# Autodesk Inventor assembly: froggy arm assm
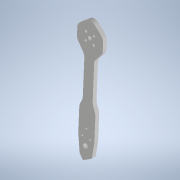
[picture p0: Inventor's stored thumbnail of the model, 180x180]
Saved by Autodesk Inventor 2020 (Build 240168000, 168)
## iProperties
Created: 2022-08-12
Part Number: froggy arm assm
Document SubType Name: Assembly
Designer: Steven
Author: Steven
## Documents named in this file (3)
- Y:\FPV drone stuff\0 Street League\Frames\experimental-quad-frames\Kauri assm\OG kauri mods\froggy arm assm.iam
- Y:\FPV drone stuff\0 Street League\Frames\experimental-quad-frames\Kauri assm\OG kauri mods\og kauri arm.ipt
- Y:\FPV drone stuff\0 Street League\Frames\experimental-quad-frames\modified Kauri arms\disc aero arms\Kauri arm disc aero.ipt
## Components (2 placed, 2 different names)
1. og kauri arm:1 — Mate:1, Mate:2, Flush:1
2. Kauri arm disc aero:1 — Mate:1, Mate:2, Flush:1
## Relationships (3: Mate 2, Flush 1)
- Mate:1: og kauri arm:1 ↔ Kauri arm disc aero:1
- Mate:2: og kauri arm:1 ↔ Kauri arm disc aero:1
- Flush:1: og kauri arm:1 ↔ Kauri arm disc aero:1
